# Autodesk Inventor assembly: Overview
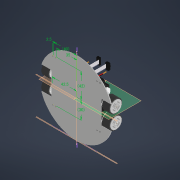
[picture p0: Inventor's stored thumbnail of the model, 180x180]
Saved by Autodesk Inventor 2022 (Build 260153000, 153)
## iProperties
Created: 2021-10-05
Part Number: Overview
Document SubType Name: Assembly
Designer: shiok
Author: shiok
## Documents named in this file (4)
- C:\Users\shiok\Documents\GitHub\Murakumo\inventor\Overview.iam
- C:\Users\shiok\Documents\GitHub\Murakumo\inventor\flame.ipt
- C:\Users\shiok\Documents\GitHub\Murakumo\inventor\Motor.iam
- C:\Users\shiok\Documents\GitHub\Murakumo\inventor\Motor_MIR.iam
## Components (3 placed, 3 different names)
1. flame:1 — メイト:1, メイト:2, フラッシュ:1, 挿入:1, 挿入:2
2. Motor:1 [sub-assembly] — メイト:6, 角度:1, 挿入:1, 挿入:2
3. Motor_MIR:1 [sub-assembly] — メイト:13, 角度:2
## Relationships (12: Mate 7, Angle 2, Insert 2, Flush 1)
- メイト:1 [Mate]: flame:1
- メイト:2 [Mate]: flame:1
- メイト:6 [Mate]: Motor:1
- メイト:7 [Mate]
- メイト:8 [Mate]
- 角度:1 [Angle] (0 deg): Motor:1
- フラッシュ:1 [Flush] (-42.5 mm): flame:1
- 挿入:1 [Insert]: flame:1 ↔ Motor:1
- 挿入:2 [Insert]: flame:1 ↔ Motor:1
- メイト:13 [Mate]: Motor_MIR:1
- メイト:14 [Mate]
- 角度:2 [Angle] (0 deg): Motor_MIR:1
